# Autodesk Inventor assembly: Arm Assembly
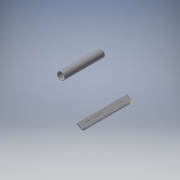
[picture p0: Inventor's stored thumbnail of the model, 180x180]
Saved by Autodesk Inventor 2016 (Build 200138000, 138)
## iProperties
Created: 2016-04-23
Part Number: Arm Assembly
Document SubType Name: Assembly
Designer: rubenjm
Author: rubenjm
## Documents named in this file (14)
- C:\Users\rubenjm\Documents\To Transfer\2k16 Spring\RME\GGC\V3\Arm Assembly.iam
- C:\Users\rubenjm\Documents\To Transfer\2k16 Spring\RME\GGC\V3\Inner Pole.ipt
- C:\Users\rubenjm\Documents\To Transfer\2k16 Spring\RME\GGC\V3\Arm Base.ipt
- C:\Users\rubenjm\Documents\To Transfer\2k16 Spring\RME\GGC\V3\Holder.ipt
- C:\Users\rubenjm\Documents\To Transfer\2k16 Spring\RME\GGC\V3\Threaded Rod Nut.ipt
- C:\Users\rubenjm\Documents\To Transfer\2k16 Spring\RME\GGC\V3\Unthreaded Rod.ipt
- C:\Users\rubenjm\Documents\To Transfer\2k16 Spring\RME\GGC\V3\Threaded Rod.ipt
- C:\Users\rubenjm\Documents\To Transfer\2k16 Spring\RME\GGC\V3\NEMA23 Motor.ipt
- C:\Users\rubenjm\Documents\To Transfer\2k16 Spring\RME\GGC\V3\Motor Coupler.ipt
- C:\Users\rubenjm\Documents\To Transfer\2k16 Spring\RME\GGC\V3\Far End Cap.ipt
- C:\Users\rubenjm\Documents\To Transfer\2k16 Spring\RME\GGC\V3\Near Holder.ipt
- C:\Users\rubenjm\Documents\To Transfer\2k16 Spring\RME\GGC\V3\Motor Bracket.ipt
- C:\Users\rubenjm\Documents\To Transfer\2k16 Spring\RME\GGC\V3\Near End Cap.ipt
- C:\Users\rubenjm\Documents\To Transfer\2k16 Spring\RME\GGC\V3\Arm Side.ipt
## Components (16 placed, 13 different names)
1. Inner Pole:1
2. Arm Base:1 — Mate:1, Mate:2, Mate:15, Mate:26, Mate:27, Flush:1, Flush:3, Mate:34, Mate:38, Flush:4, Mate:40, Flush:5, Mate:41, Mate:42, Mate:43, Mate:44, Flush:6, Flush:7
3. Holder:1 — Mate:1, Mate:2, Mate:8, Mate:9, Mate:10, Mate:12, Mate:13
4. Holder:2 — Mate:15, Mate:16, Mate:17, Mate:18, Mate:19, Mate:20
5. Threaded Rod Nut:1 — Mate:8, Mate:9, Mate:10, Mate:11
6. Threaded Rod Nut:2 — Mate:18, Mate:19, Mate:20
7. Unthreaded Rod:1 — Mate:13, Mate:16, Mate:28
8. Unthreaded Rod:2 — Mate:12, Mate:17, Mate:29
9. Threaded Rod:1 — Mate:11, Mate:24, Mate:25, Mate:30
10. NEMA23 Motor:1 — Mate:35, Mate:36, Mate:37, Mate:39
11. Motor Coupler:1 — Mate:24, Mate:25
12. Far End Cap:1 — Mate:26, Mate:27, Flush:1, Mate:28, Mate:29, Mate:30
13. Near Holder:1 — Flush:5, Mate:41, Mate:42
14. Motor Bracket:1 — Flush:3, Mate:34, Mate:35, Mate:36, Mate:37, Mate:38
15. Near End Cap:1 — Mate:39, Flush:4, Mate:40
16. Arm Side:1 — Mate:43, Mate:44, Flush:6, Flush:7
## Relationships (38: Mate 32, Flush 6)
- Mate:1: Arm Base:1 ↔ Holder:1
- Mate:2: Arm Base:1 ↔ Holder:1
- Mate:8: Holder:1 ↔ Threaded Rod Nut:1
- Mate:9: Holder:1 ↔ Threaded Rod Nut:1
- Mate:10: Holder:1 ↔ Threaded Rod Nut:1
- Mate:11: Threaded Rod Nut:1 ↔ Threaded Rod:1
- Mate:12: Holder:1 ↔ Unthreaded Rod:2
- Mate:13: Holder:1 ↔ Unthreaded Rod:1
- Mate:15: Arm Base:1 ↔ Holder:2
- Mate:16: Holder:2 ↔ Unthreaded Rod:1
- Mate:17: Holder:2 ↔ Unthreaded Rod:2
- Mate:18: Holder:2 ↔ Threaded Rod Nut:2
- Mate:19: Holder:2 ↔ Threaded Rod Nut:2
- Mate:20: Holder:2 ↔ Threaded Rod Nut:2
- Mate:24: Threaded Rod:1 ↔ Motor Coupler:1
- Mate:25: Threaded Rod:1 ↔ Motor Coupler:1
- Mate:26: Arm Base:1 ↔ Far End Cap:1
- Mate:27: Arm Base:1 ↔ Far End Cap:1
- Flush:1: Arm Base:1 ↔ Far End Cap:1
- Mate:28: Unthreaded Rod:1 ↔ Far End Cap:1
- Mate:29: Unthreaded Rod:2 ↔ Far End Cap:1
- Mate:30: Threaded Rod:1 ↔ Far End Cap:1
- Flush:3: Arm Base:1 ↔ Motor Bracket:1
- Mate:34: Arm Base:1 ↔ Motor Bracket:1
- Mate:35: NEMA23 Motor:1 ↔ Motor Bracket:1
- Mate:36: NEMA23 Motor:1 ↔ Motor Bracket:1
- Mate:37: NEMA23 Motor:1 ↔ Motor Bracket:1
- Mate:38: Arm Base:1 ↔ Motor Bracket:1
- Mate:39: NEMA23 Motor:1 ↔ Near End Cap:1
- Flush:4: Arm Base:1 ↔ Near End Cap:1
- Mate:40: Arm Base:1 ↔ Near End Cap:1
- Flush:5: Arm Base:1 ↔ Near Holder:1
- Mate:41: Arm Base:1 ↔ Near Holder:1
- Mate:42: Arm Base:1 ↔ Near Holder:1
- Mate:43: Arm Base:1 ↔ Arm Side:1
- Mate:44: Arm Base:1 ↔ Arm Side:1
- Flush:6: Arm Base:1 ↔ Arm Side:1
- Flush:7: Arm Base:1 ↔ Arm Side:1
